# Autodesk Inventor assembly: ExtruderQuickReleaseRight_MIR
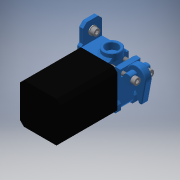
[picture p0: Inventor's stored thumbnail of the model, 180x180]
Saved by Autodesk Inventor 2016 (Build 200138000, 138)
## iProperties
Created: 2015-05-07
Part Number: ExtruderQuickReleaseRight_MIR
Document SubType Name: Assembly
Designer: Jack
Author: Jack
## Documents named in this file (14)
- C:\Users\Jack\ownCloud\Projects\CrossBot\InventorModel\Extruder\ExtruderQuickRelease\ExtruderQuickReleaseLeft.iam
- C:\Users\Jack\ownCloud\Projects\CrossBot\InventorModel\Extruder\ExtruderQuickRelease\ExtruderQuickReleaseBodyLeft.ipt
- C:\Users\Jack\ownCloud\Projects\CrossBot\InventorModel\Extruder\ExtruderQuickRelease\ExtruderQuickReleaseIdlerLeft.ipt
- C:\Users\Jack\ownCloud\Projects\CrossBot\InventorModel\Extruder\ExtruderQuickRelease\ExtruderQuickReleaseTensionCam.ipt
- C:\Users\Jack\ownCloud\Projects\CrossBot\InventorModel\Extruder\ExtruderQuickRelease\ExtruderQuickReleaseTensionDowel.ipt
- C:\Users\Jack\ownCloud\Projects\CrossBot\InventorModel\Electronics\Motors\StepperMotorNema17x60mm.ipt
- C:\Users\Jack\ownCloud\Projects\CrossBot\InventorModel\Hardware\Extruder\DriveGearMK8.ipt
- C:\Users\Jack\ownCloud\Projects\CrossBot\InventorModel\Hardware\Bearing\BearingRadialBall\BearingRadialBall624zz.ipt
- C:\Users\Jack\ownCloud\Projects\CrossBot\InventorModel\Hardware\Nuts\Nut4.ipt
- C:\Users\Jack\ownCloud\Projects\CrossBot\InventorModel\Hardware\BoltWashers\BoltWasher4\BoltWasher4x10.iam
- C:\Users\Jack\ownCloud\Projects\CrossBot\InventorModel\Hardware\Bolts\SHCS\SHCS3\SHCS3x10.ipt
- C:\Users\Jack\ownCloud\Projects\CrossBot\InventorModel\Hardware\Bolts\SHCS\SHCS3\SHCS3x20.ipt
- C:\Users\Jack\ownCloud\Projects\CrossBot\InventorModel\Hardware\Bolts\SHCS\SHCS4\SHCS4x14.ipt
- C:\Users\Jack\ownCloud\Projects\CrossBot\InventorModel\Hardware\Bolts\SHCS\SHCS4\SHCS4x40.ipt
## Components (18 placed, 13 different names)
1. ExtruderQuickReleaseBodyLeft:1 — Mate:7, Mate:6, Mate:5, Mate:4, Mate:3, Angle:2, Mate:22, Mate:32, Mate:29, Mate:31, Mate:30, Mate:17, Mate:13, Mate:16, Mate:12, Mate:15, Mate:14, Mate:24, Mate:23, Angle:3, Mate:21
2. ExtruderQuickReleaseIdlerLeft:1 — Mate:7, Mate:6, Tangent:1, Mate:9, Mate:8, Mate:11, Angle:1, Mate:19
3. ExtruderQuickReleaseTensionCam:1 — Tangent:1, Flush:2, Mate:28
4. ExtruderQuickReleaseTensionDowel:1 — Flush:2, Mate:28, Mate:33, Mate:26, Mate:34, Mate:27
5. StepperMotorNema17x60mm:1 — Mate:5, Mate:4, Mate:3, Mate:2, Mate:1
6. DriveGearMK8:1 — Mate:2, Mate:1
7. BearingRadialBall624zz:1 — Mate:9, Mate:8, Mate:10
8. Nut4:1 — Angle:2, Mate:22, Mate:25, Flush:1
9. BoltWasher4x10:1 [sub-assembly] — Mate:32, Mate:29
10. BoltWasher4x10:2 [sub-assembly] — Mate:31, Mate:30
11. SHCS3x10:1 — Mate:17, Mate:13
12. SHCS3x10:2 — Mate:16, Mate:12
13. SHCS3x20:1 — Mate:15, Mate:14
14. SHCS4x14:1 — Mate:11, Mate:10, Mate:18
15. SHCS4x40:1 — Mate:33, Mate:26, Mate:25, Mate:24, Flush:1
16. SHCS4x40:2 — Mate:34, Mate:27, Mate:23, Mate:20
17. Nut4:2 — Angle:3, Mate:21, Mate:20
18. Nut4:3 — Angle:1, Mate:19, Mate:18
## Relationships (40: Mate 34, Angle 3, Flush 2, Tangent 1)
- Mate:7 (0.2 mm): ExtruderQuickReleaseBodyLeft:1 ↔ ExtruderQuickReleaseIdlerLeft:1
- Mate:6: ExtruderQuickReleaseBodyLeft:1 ↔ ExtruderQuickReleaseIdlerLeft:1
- Tangent:1: ExtruderQuickReleaseIdlerLeft:1 ↔ ExtruderQuickReleaseTensionCam:1
- Flush:2 (-7 mm): ExtruderQuickReleaseTensionCam:1 ↔ ExtruderQuickReleaseTensionDowel:1
- Mate:28: ExtruderQuickReleaseTensionCam:1 ↔ ExtruderQuickReleaseTensionDowel:1
- Mate:5: ExtruderQuickReleaseBodyLeft:1 ↔ StepperMotorNema17x60mm:1
- Mate:4: ExtruderQuickReleaseBodyLeft:1 ↔ StepperMotorNema17x60mm:1
- Mate:3: ExtruderQuickReleaseBodyLeft:1 ↔ StepperMotorNema17x60mm:1
- Mate:2 (1 mm): StepperMotorNema17x60mm:1 ↔ DriveGearMK8:1
- Mate:1: StepperMotorNema17x60mm:1 ↔ DriveGearMK8:1
- Mate:9: ExtruderQuickReleaseIdlerLeft:1 ↔ BearingRadialBall624zz:1
- Mate:8: ExtruderQuickReleaseIdlerLeft:1 ↔ BearingRadialBall624zz:1
- Angle:2 (0 deg): ExtruderQuickReleaseBodyLeft:1 ↔ Nut4:1
- Mate:22: ExtruderQuickReleaseBodyLeft:1 ↔ Nut4:1
- Mate:32: ExtruderQuickReleaseBodyLeft:1 ↔ BoltWasher4x10:1
- Mate:29: ExtruderQuickReleaseBodyLeft:1 ↔ BoltWasher4x10:1
- Mate:31: ExtruderQuickReleaseBodyLeft:1 ↔ BoltWasher4x10:2
- Mate:30: ExtruderQuickReleaseBodyLeft:1 ↔ BoltWasher4x10:2
- Mate:17: ExtruderQuickReleaseBodyLeft:1 ↔ SHCS3x10:1
- Mate:13: ExtruderQuickReleaseBodyLeft:1 ↔ SHCS3x10:1
- Mate:16: ExtruderQuickReleaseBodyLeft:1 ↔ SHCS3x10:2
- Mate:12: ExtruderQuickReleaseBodyLeft:1 ↔ SHCS3x10:2
- Mate:15: ExtruderQuickReleaseBodyLeft:1 ↔ SHCS3x20:1
- Mate:14: ExtruderQuickReleaseBodyLeft:1 ↔ SHCS3x20:1
- Mate:11: ExtruderQuickReleaseIdlerLeft:1 ↔ SHCS4x14:1
- Mate:10: BearingRadialBall624zz:1 ↔ SHCS4x14:1
- Mate:33: ExtruderQuickReleaseTensionDowel:1 ↔ SHCS4x40:1
- Mate:26: ExtruderQuickReleaseTensionDowel:1 ↔ SHCS4x40:1
- Mate:25: Nut4:1 ↔ SHCS4x40:1
- Mate:24: ExtruderQuickReleaseBodyLeft:1 ↔ SHCS4x40:1
- Flush:1 (-2 mm): Nut4:1 ↔ SHCS4x40:1
- Mate:34: ExtruderQuickReleaseTensionDowel:1 ↔ SHCS4x40:2
- Mate:27: ExtruderQuickReleaseTensionDowel:1 ↔ SHCS4x40:2
- Mate:23: ExtruderQuickReleaseBodyLeft:1 ↔ SHCS4x40:2
- Angle:3 (0 deg): ExtruderQuickReleaseBodyLeft:1 ↔ Nut4:2
- Mate:21: ExtruderQuickReleaseBodyLeft:1 ↔ Nut4:2
- Mate:20: SHCS4x40:2 ↔ Nut4:2
- Angle:1 (0 deg): ExtruderQuickReleaseIdlerLeft:1 ↔ Nut4:3
- Mate:19: ExtruderQuickReleaseIdlerLeft:1 ↔ Nut4:3
- Mate:18: SHCS4x14:1 ↔ Nut4:3
